# Autodesk Inventor assembly: ASY 940 linkage
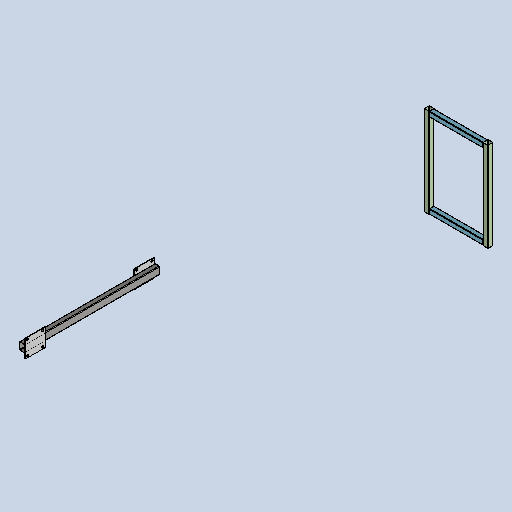
[picture p0: Inventor's stored thumbnail of the model, 512x512]
Saved by Autodesk Inventor 2025 (Build 290162010, 162A)
## iProperties
_SolveAssemblyDoc: Frame Generator Solve Assembly
_Version: 25.0.0
Created: 2024-09-11
Part Number: ASY 940 linkage
Document SubType Name: Assembly
Designer: admin
Author: admin
## Documents named in this file (5)
- C:\Users\admin\YandexDisk-badmisterfox\домашниий пк\Inventor\Manturovo\Manturovo_Se-clar\ASY 940 linkage.iam
- C:\Users\admin\YandexDisk-badmisterfox\домашниий пк\Inventor\Manturovo\Manturovo_Se-clar\Templates\Сборка рама\SKETCH рама 1.ipt
- C:\Users\admin\YandexDisk-badmisterfox\домашниий пк\Inventor\Manturovo\Manturovo_Se-clar\Templates\Сборка рама\Frame\Frame 1714907749371.iam
- C:\Users\admin\YandexDisk-badmisterfox\домашниий пк\Inventor\Manturovo\Manturovo_Se-clar\ASY MSC 900.8 base frame transverse.ipt
- C:\Users\admin\YandexDisk-badmisterfox\домашниий пк\Inventor\Manturovo\Manturovo_Se-clar\ISO 657_14 - 60x40x3 - 1000.ipt
## Components (5 placed, 4 different names)
1. SKETCH рама 1:1
2. Frame 1714907749371:1 [sub-assembly]
3. ASY MSC 900.8 base frame transverse:1
4. ASY MSC 900.8 base frame transverse:2
5. ISO 657_14 - 60x40x3 - 1000:1
## Relationships (2: WeldJoint 2)
- [WeldJoint]: ASY MSC 900.8 base frame transverse:2 ↔ ISO 657_14 - 60x40x3 - 1000:1
- [WeldJoint]: ASY MSC 900.8 base frame transverse:1 ↔ ISO 657_14 - 60x40x3 - 1000:1
